# Autodesk Inventor assembly: 446 Structural Spacer
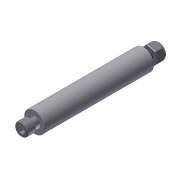
[picture p0: Inventor's stored thumbnail of the model, 180x180]
Saved by Autodesk Inventor 2013 (Build 170138000, 138)
## iProperties
Created: 2012-10-14
Part Number: 446 Structural Spacer
Document SubType Name: Assembly
Designer: Nemo
Author: Nemo
## Documents named in this file (4)
- H:\Nemo\Documents\Robotics\COTS Parts\Gearboxes\Housings\446 Structural Spacer.iam
- H:\Nemo\Documents\Robotics\COTS Parts\Fasteners\10-32 SHCS x3000.ipt
- H:\Nemo\Documents\Robotics\COTS Parts\Gearboxes\Housings\AM Shifter Spacer.ipt
- H:\Nemo\Documents\Robotics\COTS Parts\Fasteners\10-32 locknut.ipt
## Components (3 placed, 3 different names)
1. 10-32 SHCS x3000:1 — Mate:1, Mate:2, Mate:3
2. AM Shifter Spacer:1 — Mate:1, Mate:2, Mate:4
3. 10-32 locknut:1 — Mate:3, Mate:4
## Relationships (4: Mate 4)
- Mate:1: 10-32 SHCS x3000:1 ↔ AM Shifter Spacer:1
- Mate:2 (3.175 mm): 10-32 SHCS x3000:1 ↔ AM Shifter Spacer:1
- Mate:3: 10-32 SHCS x3000:1 ↔ 10-32 locknut:1
- Mate:4 (3.175 mm): AM Shifter Spacer:1 ↔ 10-32 locknut:1
